# Autodesk Inventor assembly: Disc E Assembly
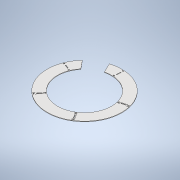
[picture p0: Inventor's stored thumbnail of the model, 180x180]
Saved by Autodesk Inventor 2020 (Build 240168000, 168)
## iProperties
Created: 2020-05-11
Part Number: Disc E Assembly
Document SubType Name: Assembly
Designer: Dan Wikman
Author: Dan Wikman
## Documents named in this file (5)
- C:\Users\Dan Wikman\OneDrive\University Life\2020, Semester 1\METR4900 Honours Thesis\Full Scale Design\Disc E Assembly.iam
- C:\Users\Dan Wikman\OneDrive\University Life\2020, Semester 1\METR4900 Honours Thesis\Full Scale Design\Platform E1.ipt
- C:\Users\Dan Wikman\OneDrive\University Life\2020, Semester 1\METR4900 Honours Thesis\Full Scale Design\Platform E2.ipt
- C:\Users\Dan Wikman\OneDrive\University Life\2020, Semester 1\METR4900 Honours Thesis\Full Scale Design\Platform E3.ipt
- C:\Users\Dan Wikman\OneDrive\University Life\2020, Semester 1\METR4900 Honours Thesis\Full Scale Design\Platform E4.ipt
## Components (4 placed, 4 different names)
1. Platform E1:1 — Flush:1, Mate:1, Mate:2
2. Platform E2:1 — Flush:1, Flush:2, Mate:1, Mate:2, Mate:3, Mate:4
3. Platform E3:1 — Flush:2, Flush:3, Mate:3, Mate:4, Mate:5, Mate:6
4. Platform E4:1 — Flush:3, Mate:5, Mate:6
## Relationships (9: Mate 6, Flush 3)
- Flush:1: Platform E1:1 ↔ Platform E2:1
- Flush:2: Platform E2:1 ↔ Platform E3:1
- Flush:3: Platform E3:1 ↔ Platform E4:1
- Mate:1: Platform E1:1 ↔ Platform E2:1
- Mate:2: Platform E1:1 ↔ Platform E2:1
- Mate:3: Platform E2:1 ↔ Platform E3:1
- Mate:4: Platform E2:1 ↔ Platform E3:1
- Mate:5: Platform E3:1 ↔ Platform E4:1
- Mate:6: Platform E3:1 ↔ Platform E4:1
